# Autodesk Inventor assembly: Unit_SR-T
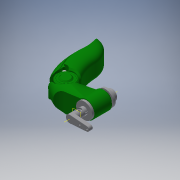
[picture p0: Inventor's stored thumbnail of the model, 180x180]
Saved by Autodesk Inventor 2019.4 (Build 234330000, 330)
## iProperties
Created: 2018-02-15
Part Number: Unit_SR-T
Material: 一般
Document SubType Name: Assembly
Designer: sktom
Author: sktom
Title: Unit_SR-T
## Documents named in this file (12)
- D:\sktometometo\Document\HACKberrySizeS_Mech\UnitHand\Unit_SR-H\Unit_SR-T\Unit_SR-T.iam
- D:\sktometometo\Document\HACKberrySizeS_Mech\UnitHand\Unit_SR-H\Unit_SR-T\SR-T-03.ipt
- D:\sktometometo\Document\HACKberrySizeS_Mech\UnitHand\Unit_SR-H\Unit_SR-T\SR-T-04.ipt
- D:\sktometometo\Document\HACKberrySizeS_Mech\UnitHand\Unit_SR-H\Unit_SR-T\SR-T-02.ipt
- D:\sktometometo\Document\HACKberrySizeS_Mech\UnitHand\Unit_SR-H\Unit_SR-T\SR-T-05.ipt
- D:\sktometometo\Document\HACKberrySizeS_Mech\UnitHand\Unit_SR-H\Unit_SR-T\SR-T-01.ipt
- D:\sktometometo\Document\HACKberrySizeS_Mech\UnitHand\Unit_SR-H\Unit_SR-T\Parts_Screw_M1.4_L6.ipt
- D:\sktometometo\Document\HACKberrySizeS_Mech\UnitHand\Unit_SR-H\Unit_SR-T\Parts_CoilSpring_CP 0.5-4.5-6.5.ipt
- D:\sktometometo\Document\HACKberrySizeS_Mech\UnitHand\Unit_SR-H\Unit_SR-T\SR-T-07.ipt
- D:\sktometometo\Document\HACKberrySizeS_Mech\UnitHand\Unit_SR-H\Unit_SR-T\SR-T-08.ipt
- D:\sktometometo\Document\HACKberrySizeS_Mech\UnitHand\Unit_SR-H\Unit_SR-T\Parts_GEF.ipt
- D:\sktometometo\Document\HACKberrySizeS_Mech\UnitHand\Unit_SR-H\Unit_SR-T\SR-T-09.ipt
## Components (14 placed, 11 different names)
1. SR-T-01 — 挿入:5, 挿入:9
2. SR-T-02 — 挿入:4, 挿入:5
3. SR-T-03 — 挿入:1, 挿入:2, 挿入:3, 挿入:4, 挿入:15, リジッド:2, フラッシュ:2, 挿入:16, 挿入:17
4. SR-T-04 — 挿入:3
5. SR-T-05 — 挿入:1, 挿入:2, 挿入:10, 挿入:11
6. SR-T-07:1 — リジッド:2, フラッシュ:1, フラッシュ:3, フラッシュ:4, フラッシュ:5, 挿入:18, 挿入:19
7. SR-T-08:1 — フラッシュ:1, フラッシュ:2
8. SR-T-09:1 — フラッシュ:3, フラッシュ:4, フラッシュ:5, 挿入:18, 挿入:19
9. Parts_GEF:2 — 挿入:17
10. Parts_GEF:1 — 挿入:16
11. Parts_CoilSpring_CP 0.5-4.5-6.5:1 — 挿入:15
12. Parts_Screw_M1.4_L6:1 — 挿入:9
13. Parts_Screw_M1.4_L6:2 — 挿入:10
14. Parts_Screw_M1.4_L6:3 — 挿入:11
## Relationships (19: Insert 13, Flush 5, WeldJoint 1)
- 挿入:1 [Insert]: SR-T-03 ↔ SR-T-05
- 挿入:2 [Insert]: SR-T-03 ↔ SR-T-05
- 挿入:3 [Insert] (1 mm): SR-T-03 ↔ SR-T-04
- 挿入:4 [Insert] (0.1 mm): SR-T-02 ↔ SR-T-03
- 挿入:5 [Insert]: SR-T-01 ↔ SR-T-02
- 挿入:9 [Insert]: SR-T-01 ↔ Parts_Screw_M1.4_L6:1
- 挿入:10 [Insert]: SR-T-05 ↔ Parts_Screw_M1.4_L6:2
- 挿入:11 [Insert]: SR-T-05 ↔ Parts_Screw_M1.4_L6:3
- 挿入:15 [Insert]: SR-T-03 ↔ Parts_CoilSpring_CP 0.5-4.5-6.5:1
- リジッド:2 [WeldJoint] (-8.9 mm): SR-T-03 ↔ SR-T-07:1
- フラッシュ:1 [Flush]: SR-T-07:1 ↔ SR-T-08:1
- フラッシュ:2 [Flush] (1 mm): SR-T-03 ↔ SR-T-08:1
- 挿入:16 [Insert]: SR-T-03 ↔ Parts_GEF:1
- 挿入:17 [Insert]: SR-T-03 ↔ Parts_GEF:2
- フラッシュ:3 [Flush]: SR-T-07:1 ↔ SR-T-09:1
- フラッシュ:4 [Flush]: SR-T-07:1 ↔ SR-T-09:1
- フラッシュ:5 [Flush]: SR-T-07:1 ↔ SR-T-09:1
- 挿入:18 [Insert]: SR-T-07:1 ↔ SR-T-09:1
- 挿入:19 [Insert]: SR-T-07:1 ↔ SR-T-09:1
